# Autodesk Inventor assembly: Assembly146-01
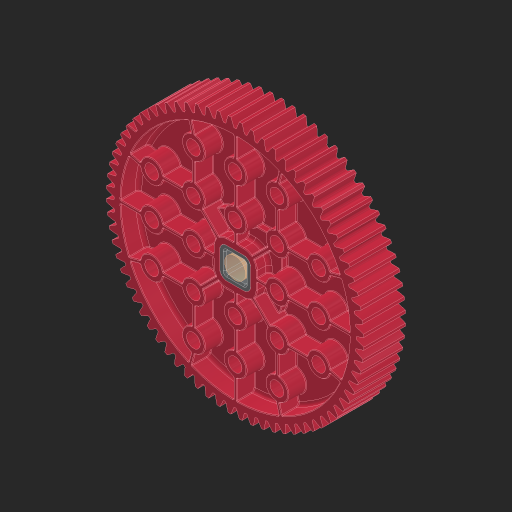
[picture p0: Inventor's stored thumbnail of the model, 512x512]
Saved by Autodesk Inventor 2023 (Build 270158000, 158)
## iProperties
Created: 2022-08-02
Part Number: Assembly146-01
Document SubType Name: Assembly
Designer: ylu12
Author: ylu12
## Documents named in this file (3)
- C:\Users\ylu12\Documents\GitHub\VEX-CAD-Inventor\Motion\Gears\HS Gear\HS 72T Gear, No Insert.iam
- C:\Users\ylu12\Documents\GitHub\VEX-CAD-Inventor\Motion\Gears\Reference Files\HS 72T Gear, No Insert.ipt
- C:\Users\ylu12\Documents\GitHub\VEX-CAD-Inventor\Motion\Gears\HS Gear.iam
## Components (1 placed, 1 different names)
1. 72T — Flush:8, Mate:15, Mate:16
## Relationships (3: Mate 2, Flush 1)
- Flush:8: 72T
- Mate:15: 72T
- Mate:16: 72T
